# Autodesk Inventor assembly: 3-22
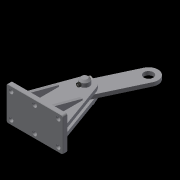
[picture p0: Inventor's stored thumbnail of the model, 180x180]
Saved by Autodesk Inventor 2017 (Build 210142000, 142)
## iProperties
Part Number: 3-22
Material: 一般
Document SubType Name: Assembly
Designer: r0909
Author: r0909
## Documents named in this file (8)
- C:\Users\r0909\Desktop\inventor\3-22.iam
- C:\Users\r0909\Desktop\inventor\3-16.ipt
- C:\Users\r0909\Desktop\inventor\3-17.ipt
- C:\Users\r0909\Desktop\inventor\3-18.ipt
- C:\Users\r0909\Desktop\inventor\3-20.ipt
- C:\Users\r0909\Desktop\inventor\3-21.ipt
- C:\Users\r0909\Desktop\inventor\3-22.1.ipt
- C:\Users\r0909\Desktop\inventor\3-22.2.ipt
## Components (11 placed, 7 different names)
1. 3-16:1 — 貼合:1, 貼合:2, 貼合:3, 貼合:5, 貼合:6, 貼合:8, 齊平:1, 貼合:11, 貼合:13, 貼合:15, 角度:2, 角度:3
2. 3-17:1 — 貼合:1, 貼合:2, 貼合:3, 貼合:4, 貼合:7, 貼合:10, 貼合:16, 貼合:17, 角度:1, 貼合:18
3. 3-18:1 — 貼合:7, 貼合:8, 齊平:1, 貼合:9, 齊平:3
4. 3-17:2 — 貼合:4, 貼合:5, 貼合:6, 貼合:12, 貼合:14, 貼合:19
5. 3-18:2 — 貼合:9, 貼合:10, 貼合:11, 齊平:2
6. 3-18:3 — 貼合:12, 貼合:13, 齊平:3
7. 3-18:4 — 貼合:14, 貼合:15, 齊平:2
8. 3-20:1 — 貼合:16, 貼合:17, 角度:1
9. 3-21:1 — 貼合:18, 貼合:19, 角度:2, 貼合:20, 相切:1, 相切:2
10. 3-22.1:1 — 貼合:20, 相切:1, 角度:3, 貼合:21, 角度:4
11. 3-22.2:1 — 貼合:21, 相切:2, 角度:4
## Relationships (30: Mate 21, Angle 4, Flush 3, Tangent 2)
- 貼合:1 [Mate]: 3-16:1 ↔ 3-17:1
- 貼合:2 [Mate]: 3-16:1 ↔ 3-17:1
- 貼合:3 [Mate] (10 mm): 3-16:1 ↔ 3-17:1
- 貼合:4 [Mate]: 3-17:1 ↔ 3-17:2
- 貼合:5 [Mate]: 3-16:1 ↔ 3-17:2
- 貼合:6 [Mate] (-30 mm): 3-16:1 ↔ 3-17:2
- 貼合:7 [Mate]: 3-17:1 ↔ 3-18:1
- 貼合:8 [Mate]: 3-16:1 ↔ 3-18:1
- 齊平:1 [Flush] (55 mm): 3-16:1 ↔ 3-18:1
- 貼合:9 [Mate] (110 mm): 3-18:1 ↔ 3-18:2
- 貼合:10 [Mate]: 3-17:1 ↔ 3-18:2
- 貼合:11 [Mate]: 3-16:1 ↔ 3-18:2
- 貼合:12 [Mate]: 3-17:2 ↔ 3-18:3
- 貼合:13 [Mate]: 3-16:1 ↔ 3-18:3
- 貼合:14 [Mate]: 3-17:2 ↔ 3-18:4
- 貼合:15 [Mate]: 3-16:1 ↔ 3-18:4
- 齊平:2 [Flush]: 3-18:2 ↔ 3-18:4
- 齊平:3 [Flush]: 3-18:1 ↔ 3-18:3
- 貼合:16 [Mate]: 3-17:1 ↔ 3-20:1
- 貼合:17 [Mate]: 3-17:1 ↔ 3-20:1
- 角度:1 [Angle] (45 deg): 3-17:1 ↔ 3-20:1
- 貼合:18 [Mate]: 3-17:1 ↔ 3-21:1
- 貼合:19 [Mate]: 3-17:2 ↔ 3-21:1
- 角度:2 [Angle] (0 deg): 3-16:1 ↔ 3-21:1
- 貼合:20 [Mate]: 3-21:1 ↔ 3-22.1:1
- 相切:1 [Tangent]: 3-21:1 ↔ 3-22.1:1
- 角度:3 [Angle] (0 deg): 3-16:1 ↔ 3-22.1:1
- 貼合:21 [Mate]: 3-22.1:1 ↔ 3-22.2:1
- 相切:2 [Tangent]: 3-21:1 ↔ 3-22.2:1
- 角度:4 [Angle] (0 deg): 3-22.1:1 ↔ 3-22.2:1
